# Autodesk Inventor assembly: WinderAssembly
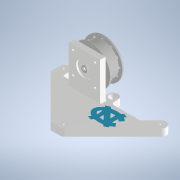
[picture p0: Inventor's stored thumbnail of the model, 180x180]
Saved by Autodesk Inventor 2020.2 (Build 242310000, 310)
## iProperties
Created: 2020-03-15
Part Number: WinderAssembly
Document SubType Name: Assembly
Designer: elmar
Author: elmar
## Documents named in this file (4)
- D:\FourWireBraidingMachine\InventorFiles\WinderAssembly.iam
- D:\FourWireBraidingMachine\InventorFiles\WinderSpool.ipt
- D:\FourWireBraidingMachine\InventorFiles\FourWireWinderBracket.ipt
- D:\FourWireBraidingMachine\InventorFiles\ShaftPlate.ipt
## Components (3 placed, 3 different names)
1. WinderSpool:1 — Insert:1
2. FourWireWinderBracket:1 — Insert:1, Insert:2
3. ShaftPlate:1 — Insert:2
## Relationships (2: Insert 2)
- Insert:1 (1 mm): WinderSpool:1 ↔ FourWireWinderBracket:1
- Insert:2 (0.5 mm): FourWireWinderBracket:1 ↔ ShaftPlate:1
